# Autodesk Inventor assembly: ServoMotor_Case
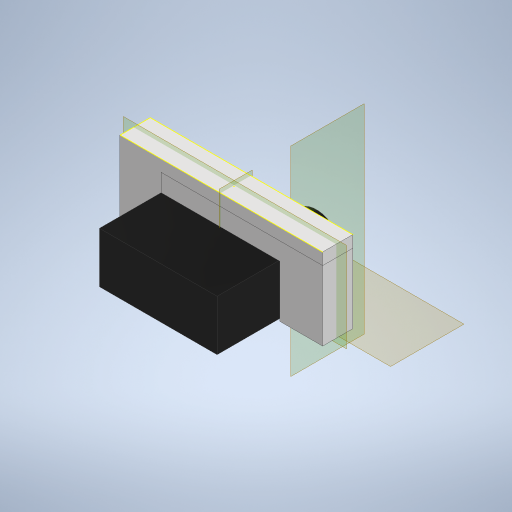
[picture p0: Inventor's stored thumbnail of the model, 512x512]
Saved by Autodesk Inventor 2024.2 (Build 282272000, 272)
## iProperties
Created: 2023-10-03
Part Number: ServoMotor_Case
Document SubType Name: Assembly
Designer: Alexander Saavedra
Author: Alexander Saavedra
## Documents named in this file (3)
- C:\Users\Laboratorio IA\Documents\handi-epn\CAD\purchased components (motors, magnets, screws, electronics)\servoMotor\ServoMotor_Case.iam
- C:\Users\Laboratorio IA\Documents\handi-epn\CAD\purchased components (motors, magnets, screws, electronics)\servoMotor Case\porta servo EPN v2.ipt
- C:\Users\Laboratorio IA\Documents\handi-epn\CAD\purchased components (motors, magnets, screws, electronics)\servoMotor\Servo.ipt
## Components (2 placed, 2 different names)
1. porta servo EPN v2:1 — Mate:1
2. Servo:1 — Mate:1
## Relationships (1: Mate 1)
- Mate:1: porta servo EPN v2:1 ↔ Servo:1
